# Autodesk Inventor assembly: a shock body
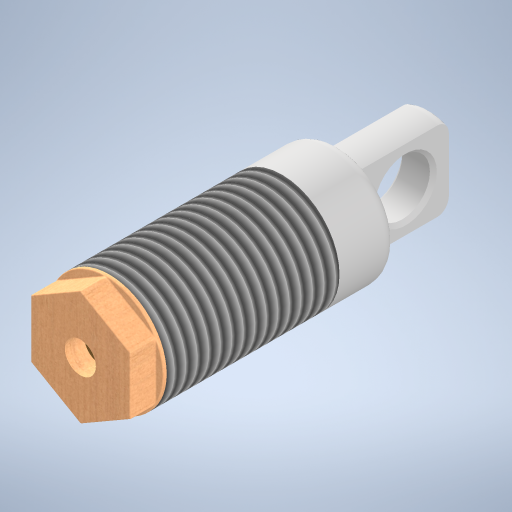
[picture p0: Inventor's stored thumbnail of the model, 512x512]
Saved by Autodesk Inventor 2024 (Build 280153000, 153)
## iProperties
Created: 2023-07-07
Part Number: a shock body
Document SubType Name: Assembly
Designer: birud
Author: birud
## Documents named in this file (3)
- C:\Users\birud\OneDrive\Desktop\Openers\a shock body.iam
- C:\Users\birud\OneDrive\Desktop\Openers\shock body 1.ipt
- C:\Users\birud\OneDrive\Desktop\Openers\a shock cartridge.iam
## Components (2 placed, 2 different names)
1. shock body 1:1 — Mate:1, Mate:2, Angle:1
2. a shock cartridge:1 [sub-assembly] — Mate:1, Mate:2, Angle:1
## Relationships (3: Mate 2, Angle 1)
- Mate:1: shock body 1:1 ↔ a shock cartridge:1
- Mate:2: shock body 1:1 ↔ a shock cartridge:1
- Angle:1 (0 deg): shock body 1:1 ↔ a shock cartridge:1
